# Autodesk Inventor assembly: 装配-载板集合终
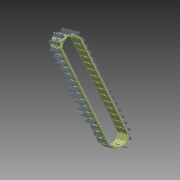
[picture p0: Inventor's stored thumbnail of the model, 180x180]
Saved by Autodesk Inventor 2015 (Build 190159000, 159)
## iProperties
Created: 2017-05-23
Part Number: 装配-载板集合终
Document SubType Name: Assembly
Designer: Administrator
Author: Administrator
## Documents named in this file (4)
- C:\Users\Administrator\Desktop\毕设改\装配-载板集合终.iam
- C:\Users\Administrator\Desktop\毕设改\装配-载板集合.iam
- C:\Users\Administrator\Desktop\毕设改\夹具右.ipt
- C:\Users\Administrator\Desktop\毕设改\夹具左.ipt
## Components (305 placed, 3 different names)
1. 装配-载板集合:1 [sub-assembly] — 插入:2, 配合:1, 配合:2, 插入:4, 角度:1, 插入:6, 角度:3, 插入:8, 角度:5, 插入:13, 配合:3, 插入:14, 配合:4, 插入:15, 角度:6, 插入:16, 角度:8, 插入:18, 角度:9, 插入:23, 角度:10, 插入:24, 角度:11, 插入:25, 角度:12, 插入:26, 角度:13, 插入:28, 角度:14, 角度:15, 插入:30, 角度:16, 角度:17, 角度:18
2. 夹具左:4 — 插入:4, 角度:2
3. 夹具右:4 — 角度:1, 角度:2
4. 夹具左:5 — 插入:6, 角度:4
5. 夹具右:5 — 角度:3, 角度:4
6. 夹具左:16 — 插入:13, 表面齐平:2
7. 夹具右:16 — 配合:3, 表面齐平:2
8. 夹具左:17 — 插入:16, 表面齐平:4
9. 夹具右:17 — 角度:8, 表面齐平:4
10. 夹具左:18 — 插入:14, 表面齐平:3
11. 夹具右:18 — 配合:4, 表面齐平:3
12. 夹具左:19 — 插入:15, 角度:7
13. 夹具右:19 — 角度:6, 角度:7
14. 夹具左:20 — 插入:18, 角度:18
15. 夹具右:20 — 角度:9
16. 夹具左:21 — 插入:23, 角度:10
17. 夹具右:21
18. 夹具左:22 — 插入:25, 角度:12
19. 夹具右:22
20. 夹具左:23 — 插入:24, 角度:11
21. 夹具右:23
22. 夹具左:42 — 插入:30, 角度:16
23. 夹具右:42 — 角度:17
24. 夹具左:44
25. 夹具右:44
26. 夹具左:45
27. 夹具右:45
28. 夹具左:46
29. 夹具右:46
30. 夹具左:47
31. 夹具右:47
32. 夹具左:48
33. 夹具右:48
34. 夹具左:49
35. 夹具右:49
36. 夹具左:50
37. 夹具右:50
38. 夹具左:51
39. 夹具右:51
40. 夹具左:52
41. 夹具右:52
42. 夹具左:53
43. 夹具右:53
44. 夹具左:54
45. 夹具右:54
46. 夹具左:82
47. 夹具右:82
48. 夹具左:83
49. 夹具右:83
50. 夹具左:84
51. 夹具右:84
52. 夹具左:85
53. 夹具右:85
54. 夹具左:86
55. 夹具右:86
56. 夹具左:87
57. 夹具右:87
58. 夹具左:88
59. 夹具右:88
60. 夹具左:89
61. 夹具右:89
62. 夹具左:90
63. 夹具右:90
64. 夹具左:91
65. 夹具右:91
66. 夹具左:92
67. 夹具右:92
68. 夹具左:120
69. 夹具右:120
70. 夹具左:121
71. 夹具右:121
72. 夹具左:122
73. 夹具右:122
74. 夹具左:123
75. 夹具右:123
76. 夹具左:124
77. 夹具右:124
78. 夹具左:125
79. 夹具右:125
80. 夹具左:126
81. 夹具右:126
82. 夹具左:127
83. 夹具右:127
84. 夹具左:128
85. 夹具右:128
86. 夹具左:129
87. 夹具右:129
88. 夹具左:130
89. 夹具右:130
90. 夹具右:1 — 插入:1, 配合:1
91. 夹具左:1 — 插入:1, 插入:2, 配合:2
92. 夹具右:2
93. 夹具左:2
94. 夹具右:3
95. 夹具左:3
96. 夹具右:6 — 表面齐平:1, 角度:5
97. 夹具左:6 — 表面齐平:1, 插入:8
98. 夹具右:7
99. 夹具左:7
100. 夹具右:8
101. 夹具左:8
102. 夹具右:9
103. 夹具左:9
104. 夹具右:10
105. 夹具左:10
106. 夹具右:43
107. 夹具左:43
108. 夹具右:24
109. 夹具左:24 — 插入:26, 角度:13
110. 夹具右:25
111. 夹具左:25
112. 夹具右:26
113. 夹具左:26
114. 夹具右:27
115. 夹具左:27
116. 夹具右:28
117. 夹具左:28
118. 夹具右:29
119. 夹具左:29
120. 夹具右:30
121. 夹具左:30
122. 夹具右:31
123. 夹具左:31
124. 夹具右:32
125. 夹具左:32
126. 夹具右:33
127. 夹具左:33
128. 夹具右:34
129. 夹具左:34
130. 夹具右:35
131. 夹具左:35
132. 夹具右:36
133. 夹具左:36
134. 夹具右:37
135. 夹具左:37
136. 夹具右:38
137. 夹具左:38
138. 夹具左:39 — 插入:28, 角度:14
139. 夹具右:39 — 角度:15
140. 夹具左:40
141. 夹具右:40
142. 夹具左:41
143. 夹具右:41
144. 夹具右:55
145. 夹具左:55
146. 夹具右:56
147. 夹具左:56
148. 夹具右:57
149. 夹具左:57
150. 夹具右:58
151. 夹具左:58
152. 夹具右:59
153. 夹具左:59
154. 夹具右:60
155. 夹具左:60
156. 夹具右:61
157. 夹具左:61
158. 夹具右:62
159. 夹具左:62
160. 夹具右:63
161. 夹具左:63
162. 夹具右:64
163. 夹具左:64
164. 夹具右:65
165. 夹具左:65
166. 夹具右:66
167. 夹具左:66
168. 夹具右:67
169. 夹具左:67
170. 夹具右:68
171. 夹具左:68
172. 夹具右:69
173. 夹具左:69
174. 夹具右:70
175. 夹具左:70
176. 夹具右:71
177. 夹具左:71
178. 夹具右:72
179. 夹具左:72
180. 夹具右:73
181. 夹具左:73
182. 夹具右:74
183. 夹具左:74
184. 夹具右:75
185. 夹具左:75
186. 夹具右:76
187. 夹具左:76
188. 夹具右:77
189. 夹具左:77
190. 夹具右:78
191. 夹具左:78
192. 夹具左:79
193. 夹具右:79
194. 夹具左:80
195. 夹具右:80
196. 夹具左:81
197. 夹具右:81
198. 夹具右:93
199. 夹具左:93
200. 夹具右:94
201. 夹具左:94
202. 夹具右:95
203. 夹具左:95
204. 夹具右:96
205. 夹具左:96
206. 夹具右:97
207. 夹具左:97
208. 夹具右:98
209. 夹具左:98
210. 夹具右:99
211. 夹具左:99
212. 夹具右:100
213. 夹具左:100
214. 夹具右:101
215. 夹具左:101
216. 夹具右:102
217. 夹具左:102
218. 夹具右:103
219. 夹具左:103
220. 夹具右:104
221. 夹具左:104
222. 夹具右:105
223. 夹具左:105
224. 夹具右:106
225. 夹具左:106
226. 夹具右:107
227. 夹具左:107
228. 夹具右:108
229. 夹具左:108
230. 夹具右:109
231. 夹具左:109
232. 夹具右:110
233. 夹具左:110
234. 夹具右:111
235. 夹具左:111
236. 夹具右:112
237. 夹具左:112
238. 夹具右:113
239. 夹具左:113
240. 夹具右:114
241. 夹具左:114
242. 夹具右:115
243. 夹具左:115
244. 夹具右:116
245. 夹具左:116
246. 夹具左:117
247. 夹具右:117
248. 夹具左:118
249. 夹具右:118
250. 夹具左:119
251. 夹具右:119
252. 夹具右:131
253. 夹具左:131
254. 夹具右:132
255. 夹具左:132
256. 夹具右:133
257. 夹具左:133
258. 夹具右:134
259. 夹具左:134
260. 夹具右:135
261. 夹具左:135
262. 夹具右:136
263. 夹具左:136
264. 夹具右:137
265. 夹具左:137
266. 夹具右:138
267. 夹具左:138
268. 夹具右:139
269. 夹具左:139
270. 夹具右:140
271. 夹具左:140
272. 夹具右:141
273. 夹具左:141
274. 夹具右:142
275. 夹具左:142
276. 夹具右:143
277. 夹具左:143
278. 夹具右:144
279. 夹具左:144
280. 夹具右:145
281. 夹具左:145
282. 夹具右:146
283. 夹具左:146
284. 夹具右:147
285. 夹具左:147
286. 夹具右:148
287. 夹具左:148
288. 夹具右:149
289. 夹具左:149
290. 夹具右:150
291. 夹具左:150
292. 夹具右:151
293. 夹具左:151
294. 夹具右:152
295. 夹具左:152
296. 夹具右:153
297. 夹具左:153
298. 夹具右:154
299. 夹具左:154
300. 夹具左:155
301. 夹具右:155
302. 夹具左:156
303. 夹具右:156
304. 夹具左:157
305. 夹具右:157
## Component patterns: (4 elements, first: 夹具左:4 + 夹具右:4 + 夹具左:5 + 夹具右:5 + 夹具左:16 + 夹具右:16 + 夹具左:17 + 夹具右:17 + 夹具左:18 + 夹具右:18 + 夹具左:19 + 夹具右:19 + 夹具左:20 + 夹具右:20 + 夹具左:21 + 夹具右:21 + 夹具左:22 + 夹具右:22 + 夹具左:23 + 夹具右:23 + 夹具左:42 + 夹具右:42), (3 elements, first: 夹具右:1 + 夹具左:1), (6 elements, first: 夹具右:6 + 夹具左:6), (15 elements, first: 夹具右:24 + 夹具左:24), (3 elements, first: 夹具左:39 + 夹具右:39), 零部件阵列 3:2 (3 elements), 零部件阵列 4:2 (6 elements), 零部件阵列 5:2 (15 elements), 零部件阵列 6:2 (3 elements), 零部件阵列 3:3 (3 elements), 零部件阵列 4:3 (6 elements), 零部件阵列 5:3 (15 elements), 零部件阵列 6:3 (3 elements), 零部件阵列 3:4 (3 elements), 零部件阵列 4:4 (6 elements), 零部件阵列 5:4 (15 elements), 零部件阵列 6:4 (3 elements)
## Relationships (60: Insert 30, Angle 18, Flush 8, Mate 4)
- 插入:1 [Insert]: 夹具右:1 ↔ 夹具左:1
- 插入:2 [Insert]: 装配-载板集合:1 ↔ 夹具左:1
- 配合:1 [Mate]: 装配-载板集合:1 ↔ 夹具右:1
- 配合:2 [Mate]: 装配-载板集合:1 ↔ 夹具左:1
- [Insert]: 夹具左:4 ↔ 夹具右:4
- 插入:4 [Insert]: 装配-载板集合:1 ↔ 夹具左:4
- 角度:1 [Angle] (-100 deg): 装配-载板集合:1 ↔ 夹具右:4
- 角度:2 [Angle] (-160 deg): 夹具左:4 ↔ 夹具右:4
- [Insert]: 夹具左:5 ↔ 夹具右:5
- 插入:6 [Insert]: 装配-载板集合:1 ↔ 夹具左:5
- 角度:3 [Angle] (-94.19 deg): 装配-载板集合:1 ↔ 夹具右:5
- 角度:4 [Angle] (-171.62 deg): 夹具左:5 ↔ 夹具右:5
- [Insert]: 夹具右:6 ↔ 夹具左:6
- 表面齐平:1 [Flush]: 夹具右:6 ↔ 夹具左:6
- 插入:8 [Insert]: 装配-载板集合:1 ↔ 夹具左:6
- 角度:5 [Angle] (-90 deg): 装配-载板集合:1 ↔ 夹具右:6
- [Insert]: 夹具左:16 ↔ 夹具右:16
- [Insert]: 夹具左:17 ↔ 夹具右:17
- [Insert]: 夹具左:18 ↔ 夹具右:18
- [Insert]: 夹具左:19 ↔ 夹具右:19
- 插入:13 [Insert]: 装配-载板集合:1 ↔ 夹具左:16
- 配合:3 [Mate]: 装配-载板集合:1 ↔ 夹具右:16
- 表面齐平:2 [Flush]: 夹具左:16 ↔ 夹具右:16
- 插入:14 [Insert]: 装配-载板集合:1 ↔ 夹具左:18
- 配合:4 [Mate]: 装配-载板集合:1 ↔ 夹具右:18
- 表面齐平:3 [Flush]: 夹具左:18 ↔ 夹具右:18
- 插入:15 [Insert]: 装配-载板集合:1 ↔ 夹具左:19
- 角度:6 [Angle] (-120 deg): 装配-载板集合:1 ↔ 夹具右:19
- 角度:7 [Angle] (-120 deg): 夹具左:19 ↔ 夹具右:19
- 插入:16 [Insert]: 装配-载板集合:1 ↔ 夹具左:17
- 角度:8 [Angle] (-90 deg): 装配-载板集合:1 ↔ 夹具右:17
- 表面齐平:4 [Flush]: 夹具左:17 ↔ 夹具右:17
- [Insert]: 夹具左:20 ↔ 夹具右:20
- 插入:18 [Insert]: 装配-载板集合:1 ↔ 夹具左:20
- 角度:9 [Angle] (-101.54 deg): 装配-载板集合:1 ↔ 夹具右:20
- [Insert]: 夹具左:21 ↔ 夹具右:21
- [Flush]: 夹具左:21 ↔ 夹具右:21
- [Insert]: 夹具左:22 ↔ 夹具右:22
- [Flush]: 夹具左:22 ↔ 夹具右:22
- [Insert]: 夹具左:23 ↔ 夹具右:23
- [Flush]: 夹具左:23 ↔ 夹具右:23
- [Insert]: 夹具右:24 ↔ 夹具左:24
- [Flush]: 夹具右:24 ↔ 夹具左:24
- 插入:23 [Insert]: 装配-载板集合:1 ↔ 夹具左:21
- 角度:10 [Angle] (-90 deg): 装配-载板集合:1 ↔ 夹具左:21
- 插入:24 [Insert]: 装配-载板集合:1 ↔ 夹具左:23
- 角度:11 [Angle] (-90 deg): 装配-载板集合:1 ↔ 夹具左:23
- 插入:25 [Insert]: 装配-载板集合:1 ↔ 夹具左:22
- 角度:12 [Angle] (-90 deg): 装配-载板集合:1 ↔ 夹具左:22
- 插入:26 [Insert]: 装配-载板集合:1 ↔ 夹具左:24
- 角度:13 [Angle] (-90 deg): 装配-载板集合:1 ↔ 夹具左:24
- [Insert]: 夹具左:39 ↔ 夹具右:39
- 插入:28 [Insert]: 装配-载板集合:1 ↔ 夹具左:39
- 角度:14 [Angle] (-101.54 deg): 装配-载板集合:1 ↔ 夹具左:39
- 角度:15 [Angle] (-101.54 deg): 装配-载板集合:1 ↔ 夹具右:39
- [Insert]: 夹具左:42 ↔ 夹具右:42
- 插入:30 [Insert]: 装配-载板集合:1 ↔ 夹具左:42
- 角度:16 [Angle] (94.19 deg): 装配-载板集合:1 ↔ 夹具左:42
- 角度:17 [Angle] (-94.19 deg): 装配-载板集合:1 ↔ 夹具右:42
- 角度:18 [Angle] (-101.54 deg): 装配-载板集合:1 ↔ 夹具左:20
## Named parameters: d50_d42 = 0 mm, d54_d42 = 0 mm, d58_d42 = 0 mm, d66_d42 = 0 mm, d67_d42 = 0 mm, d68_d42 = 0 mm, d69_d42 = 0 mm, d82_d42 = 0 mm, d86_d82_d42 = 0 mm, d87_d83 = 0 mm, d88_d82_d42 = 0 mm, d89_d83 = 0 mm, d90_d82_d42 = 0 mm, d91_d83 = 0 mm, d92_d82_d42 = 0 mm, d93_d83 = 0 mm, d106_d82_d42 = 0 mm, d115_d82_d42 = 0 mm
